# Autodesk Inventor assembly: probe-gate-with-spindel
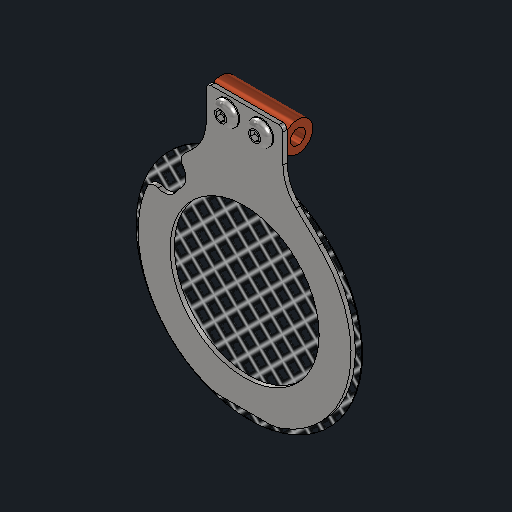
[picture p0: Inventor's stored thumbnail of the model, 512x512]
Saved by Autodesk Inventor 2026 (Build 300175050, 175E)
## iProperties
Created: 2024-05-16
Part Number: probe-gate-with-spindel
Document SubType Name: Assembly
Designer: queezz
Author: queezz
## Documents named in this file (6)
- C:\Users\queez\Dropbox\Drawings\PIHTI\Plasma Vessel\Plasma-Box\probe-gate-with-spindel.iam
- C:\Users\queez\Dropbox\Drawings\PIHTI\Plasma Vessel\Plasma-Box\probe-gate-hinge-cylinder.ipt
- C:\Users\queez\Dropbox\Drawings\PIHTI\Plasma Vessel\Plasma-Box\probe-gate.ipt
- C:\Users\queez\Dropbox\Drawings\PIHTI\ContentCenter\Fastners\M3x4-BHCS.ipt
- C:\Users\queez\Dropbox\Drawings\PIHTI\Plasma Vessel\Plasma-Box\probe-gate-mesh-circle.ipt
- C:\Users\queez\Dropbox\Drawings\PIHTI\Plasma Vessel\Plasma-Box\probe-gate-mesh-circle\probe-gate-mesh-circle-53mm.ipt
## Components (5 placed, 4 different names)
1. probe-gate-hinge-cylinder:1 — Flush:1, Flush:2, Mate:1, Mate:2, Mate:3, Mate:4
2. probe-gate:1 — Mate:2, Mate:3, Mate:4, Rotational:1, Rotational:2, Rotational:3
3. Broached Hexagon Socket Button Head Cap Screw - Metric M3 x 0.5 x 4:1 — Rotational:2
4. Broached Hexagon Socket Button Head Cap Screw - Metric M3 x 0.5 x 4:2 — Rotational:1
5. probe-gate-mesh-circle-53mm:1 — Rotational:3
## Relationships (9: Mate 4, RevoluteJoint 3, Flush 2)
- Flush:1: probe-gate-hinge-cylinder:1
- Flush:2: probe-gate-hinge-cylinder:1
- Mate:1: probe-gate-hinge-cylinder:1
- Mate:2: probe-gate-hinge-cylinder:1 ↔ probe-gate:1
- Mate:3: probe-gate-hinge-cylinder:1 ↔ probe-gate:1
- Mate:4: probe-gate-hinge-cylinder:1 ↔ probe-gate:1
- Rotational:1 [RevoluteJoint]: probe-gate:1 ↔ Broached Hexagon Socket Button Head Cap Screw - Metric M3 x 0.5 x 4:2
- Rotational:2 [RevoluteJoint]: probe-gate:1 ↔ Broached Hexagon Socket Button Head Cap Screw - Metric M3 x 0.5 x 4:1
- Rotational:3 [RevoluteJoint]: probe-gate:1 ↔ probe-gate-mesh-circle-53mm:1
